# Autodesk Inventor assembly: Złożenie testowe
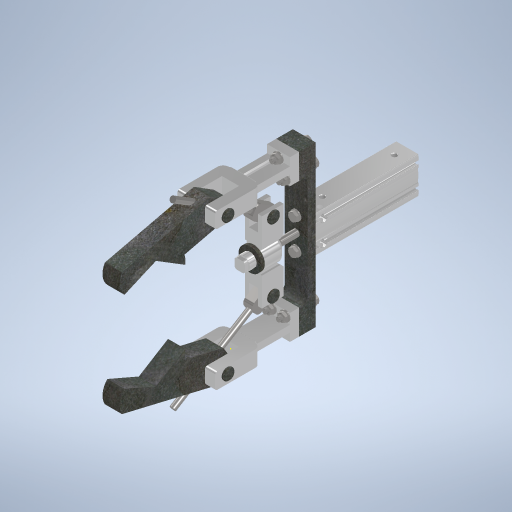
[picture p0: Inventor's stored thumbnail of the model, 512x512]
Saved by Autodesk Inventor 2024 (Build 280153000, 153)
## iProperties
Created: 2024-04-14
Part Number: Złożenie testowe
Document SubType Name: Assembly
Designer: HP
Author: HP
## Documents named in this file (29)
- C:\Users\HP\Desktop\Chwytak projekt\Złożenie testowe.iam
- C:\Users\HP\Desktop\Chwytak projekt\Siłownik.ipt
- C:\Users\HP\Desktop\Chwytak projekt\4186566 DPDM-50---(r).ipt
- C:\Users\HP\Desktop\Chwytak projekt\Belka.ipt
- C:\Users\HP\Desktop\Chwytak projekt\Mocowanie suwaka.ipt
- C:\Users\HP\Desktop\Chwytak projekt\Nakrętka na belkę.ipt
- C:\Users\HP\Desktop\Chwytak projekt\Nakrętka na tłok.ipt
- C:\Users\HP\Desktop\Chwytak projekt\Podkładka na tłok.ipt
- C:\Users\HP\Desktop\Chwytak projekt\Suwak.ipt
- C:\Users\HP\Desktop\Chwytak projekt\Rama.ipt
- C:\Users\HP\Desktop\Chwytak projekt\Uchwyt na ramę.ipt
- C:\Users\HP\Documents\Inventor\Content Center Files\R2024\en-US\ISO 7089\ISO 7089 - 4 - 140 HV(1).ipt
- C:\Users\HP\Documents\Inventor\Content Center Files\R2024\en-US\ISO 4017(1)\ISO 4017 - M4 x 16 - ISO.ipt
- C:\Users\HP\Desktop\Chwytak projekt\Ramię ze szczękami.ipt
- C:\Users\HP\Documents\Inventor\Content Center Files\R2024\en-US\ISO 4017(1)\ISO 4017 - M4 x 30 - ISO.ipt
- C:\Users\HP\Documents\Inventor\Content Center Files\R2024\en-US\ISO 4032(2)\ISO 4032 - M4 - ISO.ipt
- C:\Users\HP\Desktop\Chwytak projekt\Złożenie testowe\Design Accelerator\Clevis Pin Connection7.iam
- C:\Users\HP\Desktop\Chwytak projekt\Złożenie testowe\Design Accelerator\Clevis Pin Connection8.iam
- C:\Users\HP\Desktop\Chwytak projekt\Złożenie testowe\Design Accelerator\Clevis Pin Connection10.iam
- C:\Users\HP\Desktop\Chwytak projekt\Złożenie testowe\Design Accelerator\Clevis Pin Connection11.iam
- C:\Users\HP\Desktop\Chwytak projekt\Złożenie testowe\Design Accelerator\Clevis Pin Connection12.iam
- C:\Users\HP\Desktop\Chwytak projekt\Złożenie testowe\Design Accelerator\Clevis Pin Connection13.iam
- C:\Users\HP\Documents\Inventor\Content Center Files\R2024\en-US\ISO 1234(2)\ISO 1234 - 1,6 x 10ISO.ipt
- C:\Users\HP\Desktop\Chwytak projekt\Złożenie testowe\AIP\FEA\eo5hrb89s.fins
- C:\Users\HP\Desktop\Chwytak projekt\Złożenie testowe\AIP\FEA\eo5hrb89s.fsat
- C:\Users\HP\Desktop\Chwytak projekt\Złożenie testowe\AIP\FEA\eo5hrb89s.ftes
- C:\Users\HP\Desktop\Chwytak projekt\Złożenie testowe\AIP\FEA\eo5hrb89s.fwiz
- C:\Users\HP\Desktop\Chwytak projekt\Złożenie testowe\AIP\FEA\eo5hrb8f4.fmsh
- C:\Users\HP\Desktop\Chwytak projekt\Złożenie testowe\AIP\FEA\eo5hrb8g0.fres
## Components (51 placed, 17 different names)
1. Siłownik:1 — Cylindrical:1, Mate:2, Mate:3, Mate:4, Mate:6
2. 4186566 DPDM-50---(r):1 — Cylindrical:1, Mate:1, Rotational:1
3. Belka:1 — Rigid:1, Angle:1, Cylindrical:2, Mate:14, Rigid:3, Mate:26, Mate:27, Mate:53, Mate:54, Mate:56, Mate:57
4. Mocowanie suwaka:1 — Cylindrical:2, Mate:14, Rigid:2
5. Nakrętka na belkę:1 — Rotational:2
6. Nakrętka na tłok:1 — Rotational:1, Rigid:1
7. Podkładka na tłok:1 — Rigid:3, Rotational:2
8. Suwak:1 — Rigid:2, Cylindrical:3
9. Rama:1 — Mate:8, Mate:9, Mate:10, Angle:1, Mate:25, Mate:32, Mate:36, Mate:40, Mate:59, Mate:60, Mate:61, Mate:62
10. Uchwyt na ramę:1 — Mate:1, Mate:2, Mate:3, Mate:5, Mate:7, Mate:8, Mate:9, Mate:10, Mate:11, Mate:12, Mate:13, Mate:29, Mate:30, Mate:31, Mate:33, Mate:34, Mate:35, Mate:37, Mate:38, Mate:39, Mate:41, Mate:42, Mate:43, Mate:45, Mate:46, Mate:47, Mate:49, Mate:50, Mate:51
11. ISO 7089 4:1 — Mate:4, Mate:5, Insert:1
12. ISO 4017 M4 x 16:1 — Insert:1
13. ISO 7089 4:2 — Mate:6, Mate:7, Insert:2
14. ISO 4017 M4 x 16:2 — Insert:2
15. Rama:2 — Mate:11, Mate:12, Mate:13, Mate:28, Mate:44, Mate:48, Mate:52, Mate:63, Mate:64, Mate:65, Mate:66
16. Ramię ze szczękami:1 — Cylindrical:3, Mate:25
17. Mocowanie suwaka:2 — Rigid:4, Mate:26, Mate:27
18. Suwak:2 — Rigid:4, Cylindrical:4
19. Ramię ze szczękami:2 — Cylindrical:4, Mate:28
20. ISO 7089 4:3 — Mate:29, Mate:30, Insert:3
21. ISO 4017 M4 x 30:1 — Insert:3
22. ISO 7089 4:4 — Mate:31, Mate:32, Insert:4
23. ISO 4032 M4:1 — Insert:4
24. ISO 7089 4:5 — Mate:33, Mate:34, Insert:5
25. ISO 4017 M4 x 30:2 — Insert:5
26. ISO 7089 4:6 — Mate:35, Mate:36, Insert:6
27. ISO 4032 M4:2 — Insert:6
28. ISO 7089 4:7 — Mate:37, Mate:38, Insert:7
29. ISO 4017 M4 x 30:3 — Insert:7
30. ISO 7089 4:8 — Mate:39, Mate:40, Insert:8
31. ISO 4032 M4:3 — Insert:8
32. ISO 7089 4:9 — Mate:41, Mate:42, Insert:9
33. ISO 4017 M4 x 30:4 — Insert:9
34. ISO 7089 4:10 — Mate:43, Mate:44, Insert:10
35. ISO 4032 M4:4 — Insert:10
36. ISO 7089 4:11 — Mate:45, Mate:46, Insert:11
37. ISO 4017 M4 x 30:5 — Insert:11
38. ISO 7089 4:12 — Mate:47, Mate:48, Insert:12
39. ISO 4032 M4:5 — Insert:12
40. ISO 7089 4:13 — Mate:49, Mate:50, Insert:13
41. ISO 4017 M4 x 30:6 — Insert:13
42. ISO 7089 4:14 — Mate:51, Mate:52, Insert:14
43. ISO 4032 M4:6 — Insert:14
44. Clevis Pin Connection:1 [sub-assembly] — Mate:53, Mate:54, Rigid:6
45. Clevis Pin Connection:2 [sub-assembly] — Mate:56, Mate:57, Rigid:5
46. Clevis Pin Connection:3 [sub-assembly] — Mate:59, Mate:60
47. Clevis Pin Connection:4 [sub-assembly] — Mate:61, Mate:62
48. Clevis Pin Connection:5 [sub-assembly] — Mate:63, Mate:64
49. Clevis Pin Connection:6 [sub-assembly] — Mate:65, Mate:66
50. ISO 1234 1,6 x 10:1 — Rigid:5
51. ISO 1234 1,6 x 10:2 — Rigid:6
## Relationships (81: Mate 54, Insert 14, WeldJoint 6, CylindricalJoint 4, RevoluteJoint 2, Angle 1)
- Cylindrical:1: Siłownik:1 ↔ 4186566 DPDM-50---(r):1
- Mate:1: 4186566 DPDM-50---(r):1 ↔ Uchwyt na ramę:1
- Mate:2: Siłownik:1 ↔ Uchwyt na ramę:1
- Mate:3: Siłownik:1 ↔ Uchwyt na ramę:1
- Mate:4: Siłownik:1 ↔ ISO 7089 4:1
- Mate:5: Uchwyt na ramę:1 ↔ ISO 7089 4:1
- Insert:1: ISO 7089 4:1 ↔ ISO 4017 M4 x 16:1
- Mate:6: Siłownik:1 ↔ ISO 7089 4:2
- Mate:7: Uchwyt na ramę:1 ↔ ISO 7089 4:2
- Insert:2: ISO 7089 4:2 ↔ ISO 4017 M4 x 16:2
- Rotational:1 [RevoluteJoint]: 4186566 DPDM-50---(r):1 ↔ Nakrętka na tłok:1
- Mate:8: Rama:1 ↔ Uchwyt na ramę:1
- Mate:9: Rama:1 ↔ Uchwyt na ramę:1
- Mate:10: Rama:1 ↔ Uchwyt na ramę:1
- Mate:11: Uchwyt na ramę:1 ↔ Rama:2
- Mate:12: Uchwyt na ramę:1 ↔ Rama:2
- Mate:13: Uchwyt na ramę:1 ↔ Rama:2
- Rigid:1 [WeldJoint]: Belka:1 ↔ Nakrętka na tłok:1
- Angle:1 (0 deg): Belka:1 ↔ Rama:1
- Cylindrical:2: Belka:1 ↔ Mocowanie suwaka:1
- Mate:14: Belka:1 ↔ Mocowanie suwaka:1
- Rigid:2 [WeldJoint]: Mocowanie suwaka:1 ↔ Suwak:1
- Rigid:3 [WeldJoint]: Belka:1 ↔ Podkładka na tłok:1
- Rotational:2 [RevoluteJoint]: Nakrętka na belkę:1 ↔ Podkładka na tłok:1
- Cylindrical:3: Suwak:1 ↔ Ramię ze szczękami:1
- Mate:25: Rama:1 ↔ Ramię ze szczękami:1
- Rigid:4 [WeldJoint]: Mocowanie suwaka:2 ↔ Suwak:2
- Mate:26: Belka:1 ↔ Mocowanie suwaka:2
- Mate:27: Belka:1 ↔ Mocowanie suwaka:2
- Cylindrical:4: Suwak:2 ↔ Ramię ze szczękami:2
- Mate:28: Rama:2 ↔ Ramię ze szczękami:2
- Mate:29: Uchwyt na ramę:1 ↔ ISO 7089 4:3
- Mate:30: Uchwyt na ramę:1 ↔ ISO 7089 4:3
- Insert:3: ISO 7089 4:3 ↔ ISO 4017 M4 x 30:1
- Mate:31: Uchwyt na ramę:1 ↔ ISO 7089 4:4
- Mate:32: Rama:1 ↔ ISO 7089 4:4
- Insert:4: ISO 7089 4:4 ↔ ISO 4032 M4:1
- Mate:33: Uchwyt na ramę:1 ↔ ISO 7089 4:5
- Mate:34: Uchwyt na ramę:1 ↔ ISO 7089 4:5
- Insert:5: ISO 7089 4:5 ↔ ISO 4017 M4 x 30:2
- Mate:35: Uchwyt na ramę:1 ↔ ISO 7089 4:6
- Mate:36: Rama:1 ↔ ISO 7089 4:6
- Insert:6: ISO 7089 4:6 ↔ ISO 4032 M4:2
- Mate:37: Uchwyt na ramę:1 ↔ ISO 7089 4:7
- Mate:38: Uchwyt na ramę:1 ↔ ISO 7089 4:7
- Insert:7: ISO 7089 4:7 ↔ ISO 4017 M4 x 30:3
- Mate:39: Uchwyt na ramę:1 ↔ ISO 7089 4:8
- Mate:40: Rama:1 ↔ ISO 7089 4:8
- Insert:8: ISO 7089 4:8 ↔ ISO 4032 M4:3
- Mate:41: Uchwyt na ramę:1 ↔ ISO 7089 4:9
- Mate:42: Uchwyt na ramę:1 ↔ ISO 7089 4:9
- Insert:9: ISO 7089 4:9 ↔ ISO 4017 M4 x 30:4
- Mate:43: Uchwyt na ramę:1 ↔ ISO 7089 4:10
- Mate:44: Rama:2 ↔ ISO 7089 4:10
- Insert:10: ISO 7089 4:10 ↔ ISO 4032 M4:4
- Mate:45: Uchwyt na ramę:1 ↔ ISO 7089 4:11
- Mate:46: Uchwyt na ramę:1 ↔ ISO 7089 4:11
- Insert:11: ISO 7089 4:11 ↔ ISO 4017 M4 x 30:5
- Mate:47: Uchwyt na ramę:1 ↔ ISO 7089 4:12
- Mate:48: Rama:2 ↔ ISO 7089 4:12
- Insert:12: ISO 7089 4:12 ↔ ISO 4032 M4:5
- Mate:49: Uchwyt na ramę:1 ↔ ISO 7089 4:13
- Mate:50: Uchwyt na ramę:1 ↔ ISO 7089 4:13
- Insert:13: ISO 7089 4:13 ↔ ISO 4017 M4 x 30:6
- Mate:51: Uchwyt na ramę:1 ↔ ISO 7089 4:14
- Mate:52: Rama:2 ↔ ISO 7089 4:14
- Insert:14: ISO 7089 4:14 ↔ ISO 4032 M4:6
- Mate:53: Belka:1 ↔ Clevis Pin Connection:1
- Mate:54: Belka:1 ↔ Clevis Pin Connection:1
- Mate:56: Belka:1 ↔ Clevis Pin Connection:2
- Mate:57: Belka:1 ↔ Clevis Pin Connection:2
- Mate:59: Rama:1 ↔ Clevis Pin Connection:3
- Mate:60: Rama:1 ↔ Clevis Pin Connection:3
- Mate:61: Rama:1 ↔ Clevis Pin Connection:4
- Mate:62: Rama:1 ↔ Clevis Pin Connection:4
- Mate:63: Rama:2 ↔ Clevis Pin Connection:5
- Mate:64: Rama:2 ↔ Clevis Pin Connection:5
- Mate:65: Rama:2 ↔ Clevis Pin Connection:6
- Mate:66: Rama:2 ↔ Clevis Pin Connection:6
- Rigid:5 [WeldJoint]: Clevis Pin Connection:2 ↔ ISO 1234 1,6 x 10:1
- Rigid:6 [WeldJoint]: Clevis Pin Connection:1 ↔ ISO 1234 1,6 x 10:2
## Named parameters: sa_0 = 4560, sa_1 = 4560, sa_2 = 4560, sa_3 = 4560
note: some values were not read from the file. Shown as the stored number, unit unknown: "sa_0", "sa_1", "sa_2", "sa_3".
